# Autodesk Inventor assembly: アーム四節
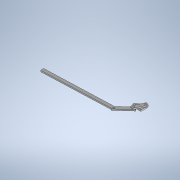
[picture p0: Inventor's stored thumbnail of the model, 180x180]
Saved by Autodesk Inventor 2020.2 (Build 242310000, 310)
## iProperties
Created: 2020-02-29
Part Number: アーム四節
Document SubType Name: Assembly
Designer: aoyam
Author: aoyam
## Documents named in this file (4)
- C:\Users\aoyam\Desktop\SRDC_local\Inventor\二年機\インナー4層丙\アーム\アーム四節.iam
- C:\Users\aoyam\Desktop\SRDC_local\Inventor\二年機\インナー3層甲\アーム中間節test.ipt
- C:\Users\aoyam\Desktop\SRDC_local\Inventor\二年機\インナー3層甲\アーム揺動節test.ipt
- C:\Users\aoyam\Desktop\SRDC_local\Inventor\二年機\インナー3層甲\アーム固定節test.ipt
## Components (3 placed, 3 different names)
1. アーム固定節test:1 — 挿入:1
2. アーム中間節test:1 — 挿入:2
3. アーム揺動節test:1 — 挿入:1, 挿入:2
## Relationships (2: Insert 2)
- 挿入:1 [Insert]: アーム固定節test:1 ↔ アーム揺動節test:1
- 挿入:2 [Insert]: アーム中間節test:1 ↔ アーム揺動節test:1
